# Autodesk Inventor assembly: noga_pre_MIR1
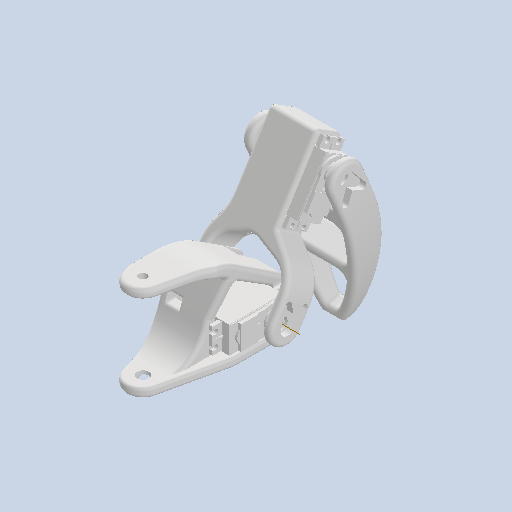
[picture p0: Inventor's stored thumbnail of the model, 512x512]
Saved by Autodesk Inventor 2023 (Build 270158000, 158)
## iProperties
Created: 2024-06-27
Part Number: noga_pre_MIR1
Document SubType Name: Assembly
Designer: kamil
Author: kamil
## Documents named in this file (8)
- C:\Users\kamil\Documents\PROJECTS - repos\Robal-2.0\mechanics\noga_pre_MIR1.iam
- C:\Users\kamil\Documents\PROJECTS - repos\Robal-2.0\mechanics\Standard-Servo_MIR3.ipt
- C:\Users\kamil\Documents\PROJECTS - repos\Robal-2.0\mechanics\blacha_dolna_pre_MIR1.ipt
- C:\Users\kamil\Documents\PROJECTS - repos\Robal-2.0\mechanics\blacha_gorna_pre_MIR1.ipt
- C:\Users\kamil\Documents\PROJECTS - repos\Robal-2.0\mechanics\uchwyt_serwa_czlon1_pre_MIR1.ipt
- C:\Users\kamil\Documents\PROJECTS - repos\Robal-2.0\mechanics\czlon2_pre_MIR2.ipt
- C:\Users\kamil\Documents\PROJECTS - repos\Robal-2.0\mechanics\czlon3_pre_MIR1.ipt
- C:\Users\kamil\Documents\PROJECTS - repos\Robal-2.0\mechanics\czlon4_pre_2_MIR1.ipt
## Components (9 placed, 7 different names)
1. Standard-Servo_MIR3:1 — Zestawiające:11, Zestawiające:10, Zestawiające:9, Zestawiające:12
2. Standard-Servo_MIR3:2 — Zestawiające:2, Równoległe:1, Zestawiające:1, Zestawiające:8, Zestawiające:7
3. blacha_dolna_pre_MIR1:1 — Zestawiające:4, Równoległe:2, Zestawiające:3
4. blacha_gorna_pre_MIR1:1 — Zestawiające:6, Równoległe:3, Zestawiające:5
5. uchwyt_serwa_czlon1_pre_MIR1:1 — Zestawiające:6, Równoległe:3, Zestawiające:5, Zestawiające:4, Równoległe:2, Zestawiające:3, Zestawiające:2, Równoległe:1, Zestawiające:1
6. czlon2_pre_MIR2:1 — Zestawiające:11, Zestawiające:10, Zestawiające:9, Zestawiające:8, Zestawiające:7, Zestawiające:13
7. czlon3_pre_MIR1:1 — Zestawiające:13, Zestawiające:12, Równoległe:4, Zestawiające:21, Zestawiające:17
8. Standard-Servo_MIR3:3 — Równoległe:4, Zestawiające:21, Zestawiające:17, Zestawiające:23, Zestawiające:22
9. czlon4_pre_2_MIR1:1 — Zestawiające:23, Zestawiające:22
## Relationships (21: Mate 17, Flush 4)
- Zestawiające:6 [Mate]: blacha_gorna_pre_MIR1:1 ↔ uchwyt_serwa_czlon1_pre_MIR1:1
- Równoległe:3 [Flush]: blacha_gorna_pre_MIR1:1 ↔ uchwyt_serwa_czlon1_pre_MIR1:1
- Zestawiające:5 [Mate]: blacha_gorna_pre_MIR1:1 ↔ uchwyt_serwa_czlon1_pre_MIR1:1
- Zestawiające:4 [Mate]: blacha_dolna_pre_MIR1:1 ↔ uchwyt_serwa_czlon1_pre_MIR1:1
- Równoległe:2 [Flush]: blacha_dolna_pre_MIR1:1 ↔ uchwyt_serwa_czlon1_pre_MIR1:1
- Zestawiające:3 [Mate]: blacha_dolna_pre_MIR1:1 ↔ uchwyt_serwa_czlon1_pre_MIR1:1
- Zestawiające:2 [Mate] (1 mm): Standard-Servo_MIR3:2 ↔ uchwyt_serwa_czlon1_pre_MIR1:1
- Równoległe:1 [Flush]: Standard-Servo_MIR3:2 ↔ uchwyt_serwa_czlon1_pre_MIR1:1
- Zestawiające:1 [Mate]: Standard-Servo_MIR3:2 ↔ uchwyt_serwa_czlon1_pre_MIR1:1
- Zestawiające:11 [Mate]: Standard-Servo_MIR3:1 ↔ czlon2_pre_MIR2:1
- Zestawiające:10 [Mate] (1 mm): Standard-Servo_MIR3:1 ↔ czlon2_pre_MIR2:1
- Zestawiające:9 [Mate] (1 mm): Standard-Servo_MIR3:1 ↔ czlon2_pre_MIR2:1
- Zestawiające:8 [Mate]: Standard-Servo_MIR3:2 ↔ czlon2_pre_MIR2:1
- Zestawiające:7 [Mate] (2.1 mm): Standard-Servo_MIR3:2 ↔ czlon2_pre_MIR2:1
- Zestawiające:13 [Mate]: czlon2_pre_MIR2:1 ↔ czlon3_pre_MIR1:1
- Zestawiające:12 [Mate] (2.1 mm): Standard-Servo_MIR3:1 ↔ czlon3_pre_MIR1:1
- Równoległe:4 [Flush]: czlon3_pre_MIR1:1 ↔ Standard-Servo_MIR3:3
- Zestawiające:21 [Mate]: czlon3_pre_MIR1:1 ↔ Standard-Servo_MIR3:3
- Zestawiające:17 [Mate] (1 mm): czlon3_pre_MIR1:1 ↔ Standard-Servo_MIR3:3
- Zestawiające:23 [Mate]: Standard-Servo_MIR3:3 ↔ czlon4_pre_2_MIR1:1
- Zestawiające:22 [Mate] (2.1 mm): Standard-Servo_MIR3:3 ↔ czlon4_pre_2_MIR1:1
